# Autodesk Inventor assembly: screw nut
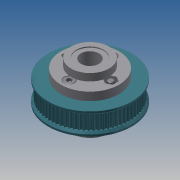
[picture p0: Inventor's stored thumbnail of the model, 180x180]
Saved by Autodesk Inventor 2013 (Build 170138000, 138)
## iProperties
Created: 2017-04-04
Part Number: screw nut
Document SubType Name: Assembly
Designer: employee
Author: employee
## Documents named in this file (7)
- C:\Users\employee\Desktop\SCARA\screw nut.iam
- C:\Users\employee\Desktop\SCARA\bearing seat 1.ipt
- C:\Users\employee\Desktop\SCARA\bearing seat 2.ipt
- C:\Users\employee\Desktop\SCARA\screw pulley.ipt
- C:\Users\employee\Desktop\SCARA\lead nut.ipt
- C:\Users\employee\Desktop\SCARA\6702.ipt
- C:\Users\employee\Desktop\SCARA\M3x18.ipt
## Components (10 placed, 6 different names)
1. bearing seat 1:1 — Mate:2, Insert:3, Insert:9, Insert:12, Insert:13
2. bearing seat 2:1 — Mate:2, Mate:3, Insert:2, Insert:8, Insert:10, Insert:11
3. screw pulley:1 — Insert:1, Mate:1, Mate:3, Insert:2, Insert:3
4. lead nut:1 — Insert:1, Mate:1
5. 6702:1 — Insert:9
6. 6702:2 — Insert:8
7. M3x18:1 — Insert:11
8. M3x18:2 — Insert:13
9. M3x18:3 — Insert:12
10. M3x18:4 — Insert:10
## Relationships (12: Insert 9, Mate 3)
- Insert:1: screw pulley:1 ↔ lead nut:1
- Mate:1: screw pulley:1 ↔ lead nut:1
- Mate:2: bearing seat 1:1 ↔ bearing seat 2:1
- Mate:3: bearing seat 2:1 ↔ screw pulley:1
- Insert:2: bearing seat 2:1 ↔ screw pulley:1
- Insert:3: bearing seat 1:1 ↔ screw pulley:1
- Insert:8: bearing seat 2:1 ↔ 6702:2
- Insert:9: bearing seat 1:1 ↔ 6702:1
- Insert:10: bearing seat 2:1 ↔ M3x18:4
- Insert:11: bearing seat 2:1 ↔ M3x18:1
- Insert:12: bearing seat 1:1 ↔ M3x18:3
- Insert:13: bearing seat 1:1 ↔ M3x18:2
